# Autodesk Inventor assembly: mechanum wheel_3
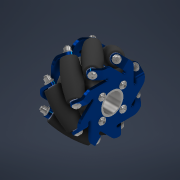
[picture p0: Inventor's stored thumbnail of the model, 180x180]
Saved by Autodesk Inventor 2021.3 (Build 253353000, 353)
## iProperties
Created: 2021-10-17
Part Number: mechanum wheel_3
Document SubType Name: Assembly
Designer: ASUS
Author: ASUS
## Documents named in this file (8)
- E:\Inventor\mecanum wheel\mechanum wheel_3.iam
- E:\Inventor\mecanum wheel\shaft.ipt
- E:\Inventor\mecanum wheel\frame.ipt
- E:\Inventor\mecanum wheel\bolt.ipt
- C:\Users\ASUS\Documents\Inventor\Content Center Files\R2021\en-US\ISO 10511\ISO 10511 - M3.ipt
- E:\Inventor\mecanum wheel\roller.ipt
- E:\Inventor\mecanum wheel\roller bracket.ipt
- E:\Inventor\mecanum wheel\roller bracket_MIR.ipt
## Components (51 placed, 7 different names)
1. shaft:1 — Mate:5, Mate:7, Mate:21, Angle:1
2. frame:1 — Mate:5, Rotational:1, Mate:15, Mate:19, Mate:20
3. frame:2 — Mate:7, Rigid:1, Mate:13, Mate:14, Mate:17
4. bolt:1 — Rigid:1
5. bolt:2
6. bolt:3
7. bolt:4
8. DIN EN ISO 10511 M3:2 — Rotational:1
9. DIN EN ISO 10511 M3:3
10. DIN EN ISO 10511 M3:4
11. DIN EN ISO 10511 M3:5
12. bolt:5 — Mate:16, Mate:17, Mate:18
13. roller:1 — Mate:9, Mate:10, Mate:11, Mate:12, Mate:14, Mate:15, Mate:16
14. roller bracket:1 — Mate:9, Mate:10, Mate:13
15. roller bracket_MIR:1 — Mate:11, Mate:12
16. DIN EN ISO 10511 M3:6 — Mate:18, Mate:20
17. bolt:6
18. roller:2
19. roller bracket:2
20. roller bracket_MIR:2
21. DIN EN ISO 10511 M3:7 — Mate:19
22. bolt:7
23. roller:3
24. roller bracket:3
25. roller bracket_MIR:3
26. DIN EN ISO 10511 M3:8
27. bolt:8
28. roller:4
29. roller bracket:4
30. roller bracket_MIR:4
31. DIN EN ISO 10511 M3:9
32. bolt:10
33. roller:6
34. roller bracket:8
35. roller bracket_MIR:5
36. DIN EN ISO 10511 M3:10
37. bolt:11
38. roller:7
39. roller bracket:9
40. roller bracket_MIR:6
41. DIN EN ISO 10511 M3:11
42. bolt:12
43. roller:8
44. roller bracket:10
45. roller bracket_MIR:7
46. DIN EN ISO 10511 M3:12
47. bolt:13
48. roller:9
49. roller bracket:11
50. roller bracket_MIR:8
51. DIN EN ISO 10511 M3:13
## Component patterns: (4 elements, first: bolt:1), (4 elements, first: DIN EN ISO 10511 M3:2), (8 elements, first: bolt:5 + roller:1 + roller bracket:1 + roller bracket_MIR:1 + DIN EN ISO 10511 M3:6)
## Relationships (18: Mate 15, WeldJoint 1, RevoluteJoint 1, Angle 1)
- Mate:5: shaft:1 ↔ frame:1
- Mate:7: shaft:1 ↔ frame:2
- Rigid:1 [WeldJoint]: frame:2 ↔ bolt:1
- Rotational:1 [RevoluteJoint]: frame:1 ↔ DIN EN ISO 10511 M3:2
- Mate:9: roller:1 ↔ roller bracket:1
- Mate:10: roller:1 ↔ roller bracket:1
- Mate:11: roller:1 ↔ roller bracket_MIR:1
- Mate:12: roller:1 ↔ roller bracket_MIR:1
- Mate:13: frame:2 ↔ roller bracket:1
- Mate:14: frame:2 ↔ roller:1
- Mate:15: frame:1 ↔ roller:1
- Mate:16: bolt:5 ↔ roller:1
- Mate:17: frame:2 ↔ bolt:5
- Mate:18: bolt:5 ↔ DIN EN ISO 10511 M3:6
- Mate:19: frame:1 ↔ DIN EN ISO 10511 M3:7
- Mate:20: frame:1 ↔ DIN EN ISO 10511 M3:6
- Mate:21: shaft:1
- Angle:1 (150 deg): shaft:1
